# Autodesk Inventor assembly: Case
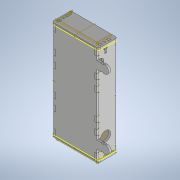
[picture p0: Inventor's stored thumbnail of the model, 180x180]
Saved by Autodesk Inventor 2020 (Build 240168000, 168)
## iProperties
Created: 2019-12-17
Part Number: Case
Document SubType Name: Assembly
Designer: erwin
Author: erwin
## Documents named in this file (9)
- D:\GitHub\ElCheapoAIS-nmea\case\Wooden Multicase\prototype\Case.iam
- D:\GitHub\ElCheapoAIS-nmea\case\Wooden Multicase\prototype\interior.ipt
- D:\GitHub\ElCheapoAIS-nmea\case\Wooden Multicase\prototype\cover.ipt
- D:\GitHub\ElCheapoAIS-nmea\case\Wooden Multicase\prototype\parameters.ipt
- D:\GitHub\ElCheapoAIS-nmea\case\Wooden Multicase\side_bottom.ipt
- D:\GitHub\ElCheapoAIS-nmea\case\Wooden Multicase\side_top.ipt
- D:\GitHub\ElCheapoAIS-nmea\case\Wooden Multicase\side_side.ipt
- D:\GitHub\ElCheapoAIS-nmea\case\Wooden Multicase\cover_components.ipt
- D:\GitHub\ElCheapoAIS-nmea\case\Wooden Multicase\cover_wires.ipt
## Components (9 placed, 8 different names)
1. interior:1 — Flush:1, Flush:2, Flush:3, Flush:4, Flush:5, Flush:6, Flush:8, Flush:9
2. cover:1 — Flush:1, Flush:2, Flush:10, Mate:1
3. parameters:1
4. side_bottom:1 — Flush:3, Flush:4, Flush:13
5. side_top:1 — Flush:5, Flush:6
6. side_side:1 — Flush:8, Flush:9
7. side_side:2 — Flush:10, Mate:1, Flush:11
8. cover_components:1 — Flush:11
9. cover_wires:1 — Flush:13
## Relationships (12: Flush 11, Mate 1)
- Flush:1: interior:1 ↔ cover:1
- Flush:2: interior:1 ↔ cover:1
- Flush:3: interior:1 ↔ side_bottom:1
- Flush:4: interior:1 ↔ side_bottom:1
- Flush:5: interior:1 ↔ side_top:1
- Flush:6: interior:1 ↔ side_top:1
- Flush:8: interior:1 ↔ side_side:1
- Flush:9: interior:1 ↔ side_side:1
- Flush:10: cover:1 ↔ side_side:2
- Mate:1: cover:1 ↔ side_side:2
- Flush:11: side_side:2 ↔ cover_components:1
- Flush:13: side_bottom:1 ↔ cover_wires:1
